# Autodesk Inventor assembly: Сборка3
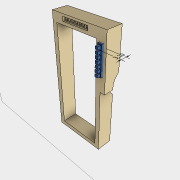
[picture p0: Inventor's stored thumbnail of the model, 180x180]
Saved by Autodesk Inventor 2021.2 (Build 252289000, 289)
## iProperties
Created: 2025-10-29
Part Number: Сборка3
Document SubType Name: Assembly
Designer: Захаров
Author: Захаров
## Documents named in this file (3)
- C:\Users\User\Documents\CaseARHead1\Сборка3.iam
- C:\Users\User\Documents\CaseARHead1\ЛЦМК000002.00.00.00.00.06-01.ipt
- C:\Users\User\Documents\CaseARHead1\ЛЦМК.00002.00.00.00.00.01.ipt
## Components (2 placed, 2 different names)
1. ЛЦМК000002.00.00.00.00.06-01:1 — Заподлицо:1, Совмещение:1, Заподлицо:2
2. ЛЦМК.00002.00.00.00.00.01:1 — Заподлицо:1, Совмещение:1, Заподлицо:2
## Relationships (3: Flush 2, Mate 1)
- Заподлицо:1 [Flush] (-3.2 mm): ЛЦМК000002.00.00.00.00.06-01:1 ↔ ЛЦМК.00002.00.00.00.00.01:1
- Совмещение:1 [Mate] (1 mm): ЛЦМК000002.00.00.00.00.06-01:1 ↔ ЛЦМК.00002.00.00.00.00.01:1
- Заподлицо:2 [Flush] (1.8 mm): ЛЦМК000002.00.00.00.00.06-01:1 ↔ ЛЦМК.00002.00.00.00.00.01:1
